# Autodesk Inventor assembly: Cell stretcher assembly
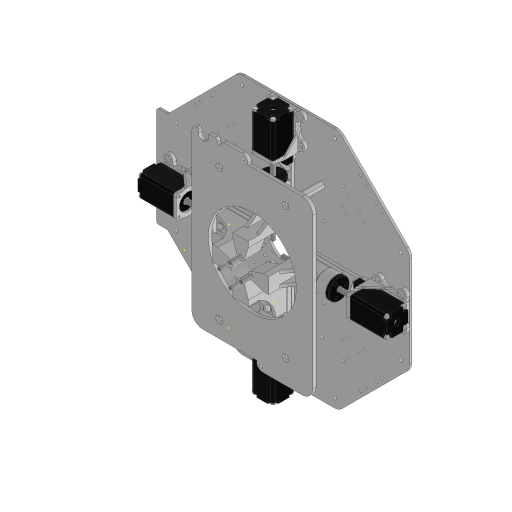
[picture p0: Inventor's stored thumbnail of the model, 512x512]
Saved by Autodesk Inventor 2023 (Build 270158000, 158)
## iProperties
Created: 2022-03-01
Part Number: Cell stretcher assembly
Document SubType Name: Assembly
Designer: ferrerx
Author: ferrerx
## Documents named in this file (6)
- C:\Users\ferrerx\Documents\GitHub\Cell_stretcher_8DOF\Design files\Mechanics V2\Cell stretcher assembly.iam
- C:\Users\ferrerx\Documents\GitHub\Cell_stretcher_8DOF\Design files\Mechanics V2\Base.ipt
- C:\Users\ferrerx\Documents\GitHub\Cell_stretcher_8DOF\Design files\Mechanics V2\Linear actuator.iam
- C:\Users\ferrerx\Documents\GitHub\Cell_stretcher_8DOF\Design files\Mechanics V2\Microscope lid.ipt
- C:\Users\ferrerx\Documents\GitHub\Cell_stretcher_8DOF\Design files\Mechanics V2\Electronics spacer.ipt
- C:\Users\ferrerx\Documents\GitHub\Cell_stretcher_8DOF\Four actuator mould\PDMS_insert.ipt
## Components (9 placed, 5 different names)
1. Base:1 — Mate:1, Mate:2, Mate:16, Mate:17, Mate:19, Mate:20, Mate:25, Mate:26, Mate:51, Mate:52, Mate:54, Mate:56, Mate:57, Mate:58, Mate:59, Mate:60, Mate:63, Mate:65
2. Linear actuator:1 [sub-assembly] — Mate:1, Mate:2, Mate:59, Mate:64
3. Linear actuator:7 [sub-assembly] — Mate:16, Mate:17, Mate:60
4. Linear actuator:8 [sub-assembly] — Mate:19, Mate:20, Mate:58
5. Linear actuator:9 [sub-assembly] — Mate:25, Mate:26, Mate:57
6. Microscope lid:1 — Mate:51, Mate:52, Mate:61, Mate:62
7. Electronics spacer:1 — Mate:54, Mate:62, Mate:63
8. Electronics spacer:4 — Mate:56, Mate:61
9. PDMS_insert:1 — Mate:64
## Relationships (21: Mate 21)
- Mate:1: Base:1 ↔ Linear actuator:1
- Mate:2: Base:1 ↔ Linear actuator:1
- Mate:16: Base:1 ↔ Linear actuator:7
- Mate:17: Base:1 ↔ Linear actuator:7
- Mate:19: Base:1 ↔ Linear actuator:8
- Mate:20: Base:1 ↔ Linear actuator:8
- Mate:25: Base:1 ↔ Linear actuator:9
- Mate:26: Base:1 ↔ Linear actuator:9
- Mate:51: Base:1 ↔ Microscope lid:1
- Mate:52: Base:1 ↔ Microscope lid:1
- Mate:54: Base:1 ↔ Electronics spacer:1
- Mate:56: Base:1 ↔ Electronics spacer:4
- Mate:57: Base:1 ↔ Linear actuator:9
- Mate:58: Base:1 ↔ Linear actuator:8
- Mate:59: Base:1 ↔ Linear actuator:1
- Mate:60: Base:1 ↔ Linear actuator:7
- Mate:61: Microscope lid:1 ↔ Electronics spacer:4
- Mate:62: Microscope lid:1 ↔ Electronics spacer:1
- Mate:63: Base:1 ↔ Electronics spacer:1
- Mate:64: Linear actuator:1 ↔ PDMS_insert:1
- Mate:65: Base:1
